# Autodesk Inventor assembly: GripperSidePlate
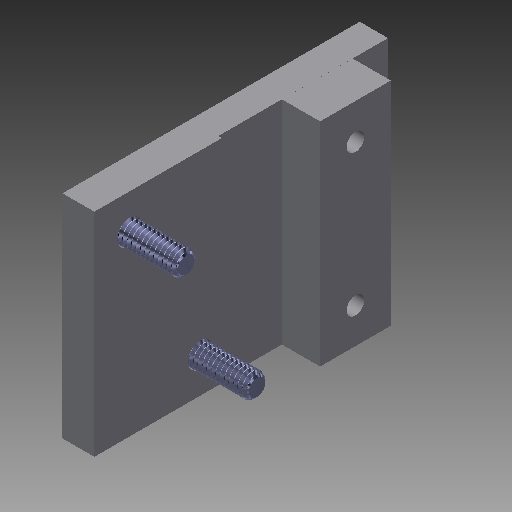
[picture p0: Inventor's stored thumbnail of the model, 512x512]
Saved by Autodesk Inventor 2019 (Build 230136000, 136)
## iProperties
Created: 2019-10-03
Part Number: GripperSidePlate
Document SubType Name: Assembly
Designer: james
Author: james
## Documents named in this file (5)
- F:\JimsDesign\Jims2020FTC\GripperSidePlate.iam
- F:\JimsDesign\Jims2020FTC\GripperSidePlate.ipt
- F:\JimsDesign\Library\McMaster\Screws\91771A196_18-8 SS FLAT HEAD PHILLIPS MACHINE SCREW.ipt
- F:\JimsDesign\Library\McMaster\Screws\91771A192_18-8 SS FLAT HEAD PHILLIPS MACHINE SCREW.ipt
- F:\JimsDesign\Jims2020FTC\GripperSliderBlock.ipt
## Components (6 placed, 4 different names)
1. GripperSidePlate:1 — Mate:1, Mate:2, Mate:3, Mate:4, Flush:1, Flush:2, Flush:3, Flush:4, Mate:5
2. 91771A196_18-8 SS FLAT HEAD PHILLIPS MACHINE SCREW:1 — Mate:3, Flush:1
3. 91771A196_18-8 SS FLAT HEAD PHILLIPS MACHINE SCREW:2 — Mate:4, Flush:2
4. 91771A192_18-8 SS FLAT HEAD PHILLIPS MACHINE SCREW:1 — Mate:2, Flush:4, Mate:6
5. 91771A192_18-8 SS FLAT HEAD PHILLIPS MACHINE SCREW:2 — Mate:1, Flush:3, Mate:7
6. GripperSliderBlock:1 — Mate:5, Mate:6, Mate:7
## Relationships (11: Mate 7, Flush 4)
- Mate:1: GripperSidePlate:1 ↔ 91771A192_18-8 SS FLAT HEAD PHILLIPS MACHINE SCREW:2
- Mate:2: GripperSidePlate:1 ↔ 91771A192_18-8 SS FLAT HEAD PHILLIPS MACHINE SCREW:1
- Mate:3: GripperSidePlate:1 ↔ 91771A196_18-8 SS FLAT HEAD PHILLIPS MACHINE SCREW:1
- Mate:4: GripperSidePlate:1 ↔ 91771A196_18-8 SS FLAT HEAD PHILLIPS MACHINE SCREW:2
- Flush:1: GripperSidePlate:1 ↔ 91771A196_18-8 SS FLAT HEAD PHILLIPS MACHINE SCREW:1
- Flush:2: GripperSidePlate:1 ↔ 91771A196_18-8 SS FLAT HEAD PHILLIPS MACHINE SCREW:2
- Flush:3: GripperSidePlate:1 ↔ 91771A192_18-8 SS FLAT HEAD PHILLIPS MACHINE SCREW:2
- Flush:4: GripperSidePlate:1 ↔ 91771A192_18-8 SS FLAT HEAD PHILLIPS MACHINE SCREW:1
- Mate:5: GripperSidePlate:1 ↔ GripperSliderBlock:1
- Mate:6: 91771A192_18-8 SS FLAT HEAD PHILLIPS MACHINE SCREW:1 ↔ GripperSliderBlock:1
- Mate:7: 91771A192_18-8 SS FLAT HEAD PHILLIPS MACHINE SCREW:2 ↔ GripperSliderBlock:1
